# Autodesk Inventor assembly: Клиновая передача
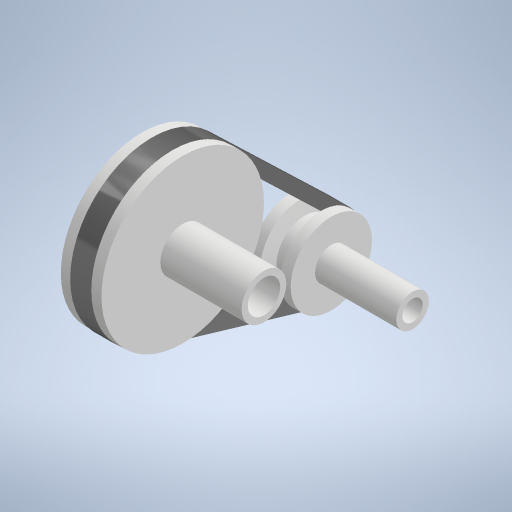
[picture p0: Inventor's stored thumbnail of the model, 512x512]
Saved by Autodesk Inventor 2023 (Build 270158000, 158)
## iProperties
Created: 2022-05-13
Part Number: Клиновая передача
Document SubType Name: Assembly
Designer: avkap
Author: avkap
## Documents named in this file (4)
- D:\Стойка\VR-simulator-3D-models\Механизм\Клиновая передача.iam
- D:\Стойка\VR-simulator-3D-models\Механизм\Шкив 20.ipt
- D:\Стойка\VR-simulator-3D-models\Механизм\Шкив 80.ipt
- D:\Стойка\VR-simulator-3D-models\Механизм\Клиновая передача\Мастер проектирования\Передача клиновым ремнем1.iam
## Components (3 placed, 3 different names)
1. Шкив 20:1 — Заподлицо:1
2. Шкив 80:1 — Заподлицо:1
3. Передача клиновым ремнем:1 [sub-assembly]
## Relationships (1: Flush 1)
- Заподлицо:1 [Flush]: Шкив 20:1 ↔ Шкив 80:1
